# Autodesk Inventor assembly: MainV2
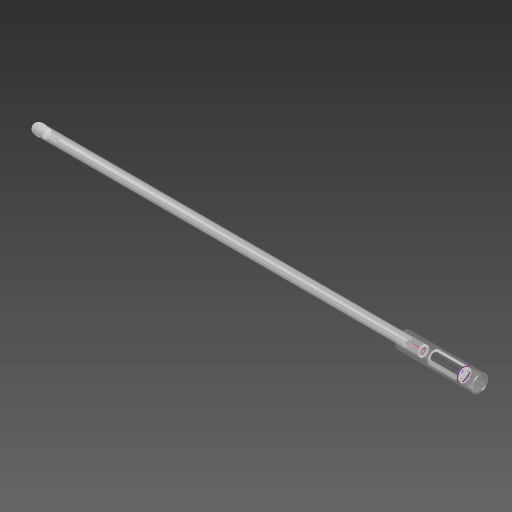
[picture p0: Inventor's stored thumbnail of the model, 512x512]
Saved by Autodesk Inventor 2023.1 (Build 271208000, 208)
## iProperties
Manager: N/A
Company: N/A
Created: 2022-02-04
Part Number: MainV2
Document SubType Name: Assembly
Designer: Michael Lacey
Mass: 1181.48 g
Surface Area: 4169 cm^2
Volume: 721.445 cm^3
Density: 1.63766 g/cm^3
Engineer: Michael Lacey
Author: Michael Lacey
Title: Full Light Saber Assembly
Subject: LightSaber Prop
## Documents named in this file (5)
- C:\Users\foams\OneDrive\3D Objects\Light Saber\All Files Compiled\CAD\MainV2.iam
- C:\Users\foams\OneDrive\3D Objects\Light Saber\All Files Compiled\CAD\Blade Assembly.iam
- C:\Users\foams\OneDrive\3D Objects\Light Saber\All Files Compiled\CAD\MainHilt.ipt
- C:\Users\foams\OneDrive\3D Objects\Light Saber\Battery.ipt
- C:\Users\foams\OneDrive\3D Objects\Light Saber\All Files Compiled\BatteryHolder.ipt
## Components (4 placed, 4 different names)
1. MainHilt:1 — Mate:15, Mate:16
2. Blade Assembly:1 [sub-assembly]
3. Battery:1 — Tangent:1, Tangent:2, Mate:14
4. BatteryHolder:1 — Tangent:1, Tangent:2, Mate:14, Mate:15, Mate:16
## Relationships (7: Mate 5, Tangent 2)
- [Mate]: MainHilt:1 ↔ Blade Assembly:1
- [Mate]: MainHilt:1 ↔ Blade Assembly:1
- Tangent:1: Battery:1 ↔ BatteryHolder:1
- Tangent:2: Battery:1 ↔ BatteryHolder:1
- Mate:14: Battery:1 ↔ BatteryHolder:1
- Mate:15: MainHilt:1 ↔ BatteryHolder:1
- Mate:16: MainHilt:1 ↔ BatteryHolder:1
